# Autodesk Inventor assembly: kayboard
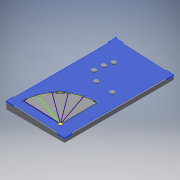
[picture p0: Inventor's stored thumbnail of the model, 180x180]
Saved by Autodesk Inventor 2016 SP2 (Build 200236200, 236)
## iProperties
Created: 2017-09-03
Part Number: kayboard
Document SubType Name: Assembly
Designer: Kartikye
Author: Kartikye
## Documents named in this file (8)
- C:\Users\Kartikye\OneDrive\Documents\class\cs294\TextEntryDevice\CAD\keyboard.iam
- C:\Users\Kartikye\OneDrive\Documents\class\cs294\TextEntryDevice\CAD\main_plate.ipt
- C:\Users\Kartikye\OneDrive\Documents\class\cs294\TextEntryDevice\CAD\swiveller.ipt
- C:\Users\Kartikye\OneDrive\Documents\class\cs294\TextEntryDevice\CAD\side_plate.ipt
- C:\Users\Kartikye\OneDrive\Documents\class\cs294\TextEntryDevice\CAD\bottom_plate.ipt
- C:\Users\Kartikye\OneDrive\Documents\class\cs294\TextEntryDevice\CAD\button.iam
- C:\Users\Kartikye\OneDrive\Documents\class\cs294\TextEntryDevice\CAD\back_plate.ipt
- C:\Users\Kartikye\OneDrive\Documents\class\cs294\TextEntryDevice\CAD\front_plate.ipt
## Components (12 placed, 7 different names)
1. swiveller:1 — Insert:1
2. main_plate:1 — Insert:1, Mate:1, Flush:1, Mate:2, Mate:3, Flush:2, Mate:4, Insert:2, Insert:3, Insert:4, Insert:5, Insert:6
3. side_plate:1 — Mate:1, Flush:1, Mate:2
4. side_plate:2 — Mate:3, Flush:2, Mate:4, Mate:5, Flush:3, Mate:6
5. bottom_plate:1 — Mate:5, Flush:3, Mate:6, Mate:7, Mate:8, Mate:9, Mate:10, Mate:11, Mate:12
6. button:1 [sub-assembly] — Insert:5
7. button:2 [sub-assembly] — Insert:6
8. button:3 [sub-assembly] — Insert:4
9. button:4 [sub-assembly] — Insert:3
10. button:5 [sub-assembly] — Insert:2
11. back_plate:1 — Mate:7, Mate:8, Mate:9
12. front_plate:1 — Mate:10, Mate:11, Mate:12
## Relationships (21: Mate 12, Insert 6, Flush 3)
- Insert:1: swiveller:1 ↔ main_plate:1
- Mate:1: main_plate:1 ↔ side_plate:1
- Flush:1: main_plate:1 ↔ side_plate:1
- Mate:2: main_plate:1 ↔ side_plate:1
- Mate:3: main_plate:1 ↔ side_plate:2
- Flush:2: main_plate:1 ↔ side_plate:2
- Mate:4: main_plate:1 ↔ side_plate:2
- Mate:5: side_plate:2 ↔ bottom_plate:1
- Flush:3: side_plate:2 ↔ bottom_plate:1
- Mate:6: side_plate:2 ↔ bottom_plate:1
- Insert:2: main_plate:1 ↔ button:5
- Insert:3: main_plate:1 ↔ button:4
- Insert:4: main_plate:1 ↔ button:3
- Insert:5: main_plate:1 ↔ button:1
- Insert:6: main_plate:1 ↔ button:2
- Mate:7: bottom_plate:1 ↔ back_plate:1
- Mate:8: bottom_plate:1 ↔ back_plate:1
- Mate:9: bottom_plate:1 ↔ back_plate:1
- Mate:10: bottom_plate:1 ↔ front_plate:1
- Mate:11: bottom_plate:1 ↔ front_plate:1
- Mate:12: bottom_plate:1 ↔ front_plate:1
